# Autodesk Inventor assembly: forkMountForDecTripV03
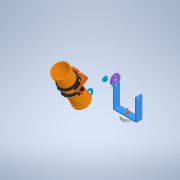
[picture p0: Inventor's stored thumbnail of the model, 180x180]
Saved by Autodesk Inventor 2021.2 (Build 252289000, 289)
## iProperties
Created: 2020-11-06
Part Number: forkMountForDecTripV03
Document SubType Name: Assembly
Designer: robst
Mass: 4855.93 g
Surface Area: 5697.22 cm^2
Volume: 1885.92 cm^3
Density: 2.57483 g/cm^3
Author: robst
## Documents named in this file (13)
- C:\git\CAD-Development\robSteele\ShapeWays\TelescopeProjects\TelescopeMount\forkMountForDecTripV03.iam
- C:\git\CAD-Development\robSteele\ShapeWays\TelescopeProjects\TelescopeMount\telescopeTube.ipt
- C:\git\CAD-Development\robSteele\ShapeWays\TelescopeProjects\TelescopeMount\celestronTubeBracket.ipt
- C:\git\CAD-Development\robSteele\ShapeWays\TelescopeProjects\TelescopeMount\connectorToTubeBrackeCradle.ipt
- C:\git\CAD-Development\robSteele\ShapeWays\TelescopeProjects\TelescopeMount\forkV03.ipt
- C:\git\CAD-Development\robSteele\ShapeWays\TelescopeProjects\TelescopeMount\forkMountForDecTripV01\Design Accelerator\Worm Gears5.iam
- C:\git\CAD-Development\robSteele\ShapeWays\TelescopeProjects\TelescopeMount\SplineLock\centerPartOfLock.ipt
- C:\git\CAD-Development\robSteele\ShapeWays\TelescopeProjects\TelescopeMount\SplineLock\outerPartOfLock.ipt
- C:\git\CAD-Development\robSteele\ShapeWays\TelescopeProjects\TelescopeMount\1_2x3-inchHexShaft_MIR.ipt
- C:\git\CAD-Development\robSteele\ShapeWays\TelescopeProjects\TelescopeMount\baseSupport.ipt
- C:\git\CAD-Development\robSteele\ShapeWays\TelescopeProjects\TelescopeMount\3_8x5_8-hexBearing.ipt
- C:\git\CAD-Development\robSteele\ShapeWays\TelescopeProjects\TelescopeMountNov2020\1_2x3-inchHexShaft.ipt
- C:\git\CAD-Development\robSteele\ShapeWays\TelescopeProjects\TelescopeMountNov2020\3_8x3-inchHexShaft.ipt
## Components (17 placed, 12 different names)
1. telescopeTube:1 — Insert:1, Flush:3
2. connectorToTubeBrackeCradle:1 — Mate:10, Mate:11, Mate:12, Mate:13, Mate:14, Mate:15, Mate:16, Mate:17, Mate:18, Flush:4
3. celestronTubeBracket:1 — Insert:1, Mate:13, Mate:14, Mate:15
4. celestronTubeBracket:2 — Mate:10, Mate:11, Mate:12
5. forkV03:1 — Flush:1, Flush:2, Mate:19, Flush:5, Flush:6, Flush:7, Mate:20, Flush:8, Flush:9, Flush:10
6. Worm Gears:1 [sub-assembly]
7. centerPartOfLock:1
8. outerPartOfLock:1
9. 1_2x3-inchHexShaft:3 — Mate:16, Mate:17, Mate:18
10. 1_2x3-inchHexShaft_MIR:1
11. centerPartOfLock:2 — Insert:2
12. Worm Gears:2 [sub-assembly] — Flush:7, Mate:20, Flush:8, Insert:2, Mate:21, Mate:22
13. 1_2x3-inchHexShaft:4 — Mate:19, Flush:5, Flush:6
14. outerPartOfLock:2 — Mate:21
15. baseSupport:1 — Flush:9, Flush:10
16. 3_8x3-inchHexShaft:1 — Mate:22
17. 3_8x5_8-hexBearing:1
## Relationships (25: Mate 13, Flush 10, Insert 2)
- Insert:1 (203.2 mm): telescopeTube:1 ↔ celestronTubeBracket:1
- Mate:10: connectorToTubeBrackeCradle:1 ↔ celestronTubeBracket:2
- Mate:11: connectorToTubeBrackeCradle:1 ↔ celestronTubeBracket:2
- Mate:12: connectorToTubeBrackeCradle:1 ↔ celestronTubeBracket:2
- Mate:13: connectorToTubeBrackeCradle:1 ↔ celestronTubeBracket:1
- Mate:14: connectorToTubeBrackeCradle:1 ↔ celestronTubeBracket:1
- Mate:15: connectorToTubeBrackeCradle:1 ↔ celestronTubeBracket:1
- Flush:1: forkV03:1
- Flush:2: forkV03:1
- Mate:16: connectorToTubeBrackeCradle:1 ↔ 1_2x3-inchHexShaft:3
- Mate:17: connectorToTubeBrackeCradle:1 ↔ 1_2x3-inchHexShaft:3
- Mate:18: connectorToTubeBrackeCradle:1 ↔ 1_2x3-inchHexShaft:3
- Flush:3: telescopeTube:1
- Flush:4: connectorToTubeBrackeCradle:1
- Mate:19: forkV03:1 ↔ 1_2x3-inchHexShaft:4
- Flush:5: forkV03:1 ↔ 1_2x3-inchHexShaft:4
- Flush:6: forkV03:1 ↔ 1_2x3-inchHexShaft:4
- Flush:7: forkV03:1 ↔ Worm Gears:2
- Mate:20 (6.35 mm): forkV03:1 ↔ Worm Gears:2
- Flush:8: forkV03:1 ↔ Worm Gears:2
- Insert:2: centerPartOfLock:2 ↔ Worm Gears:2
- Mate:21: Worm Gears:2 ↔ outerPartOfLock:2
- Flush:9: forkV03:1 ↔ baseSupport:1
- Flush:10: forkV03:1 ↔ baseSupport:1
- Mate:22: Worm Gears:2 ↔ 3_8x3-inchHexShaft:1
